# Autodesk Inventor assembly: ARM_012_ArmMount
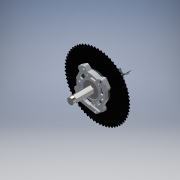
[picture p0: Inventor's stored thumbnail of the model, 180x180]
Saved by Autodesk Inventor 2018.3 (Build 223284000, 284)
## iProperties
Created: 2020-01-31
Part Number: ARM_012_ArmMount
Document SubType Name: Assembly
Designer: 21vogecale
Author: 21vogecale
## Documents named in this file (7)
- C:\Users\21vogecale\Documents\GrabCAD\Infinite Recharge 2020\Build season\ARM_012_ArmMount.iam
- C:\Users\21vogecale\Documents\GrabCAD\Deep Space 2019\Build Season\Brainstorming\End effector (hatches)\_64t_Aluminum_Plate_Sprocket_25_Chain_1-1_8_Bearing_Bore_217-2629.ipt
- C:\Users\21vogecale\Documents\GrabCAD\Deep Space 2019\Build Season\Brainstorming\End effector (hatches)\Arm plastic VersaHub.ipt
- C:\Users\21vogecale\Documents\GrabCAD\Deep Space 2019\Build Season\Chassis\217-2731_0_500_flanged_bearing.ipt
- C:\Users\21vogecale\Documents\GrabCAD\Deep Space 2019\Build Season\Master references\VersaBlock_V2_217-6111.ipt
- C:\Users\21vogecale\Documents\GrabCAD\Deep Space 2019\Build Season\Brainstorming\End effector (hatches)\Arm Pivot Hex Shaft.ipt
- C:\Users\21vogecale\Documents\GrabCAD\Infinite Recharge 2020\Brainstorming\Sam's Brainstorming Folder\Bearing Mount.ipt
## Components (7 placed, 6 different names)
1. _64t_Aluminum_Plate_Sprocket_25_Chain_1-1_8_Bearing_Bore_217-2629:1 — Insert:2, Mate:7, Mate:11
2. Arm plastic VersaHub:1 — Insert:2, Mate:7, Insert:3, Mate:8
3. 217-2731_0_500_flanged_bearing:2 — Mate:5, Mate:6, Mate:10
4. VersaBlock_V2_217-6111:1 — Mate:5, Mate:6, Insert:3, Mate:8
5. Arm Pivot Hex Shaft:1 — Insert:1, Mate:10
6. 217-2731_0_500_flanged_bearing:3 — Mate:1, Mate:2, Insert:1
7. Bearing Mount:1 — Mate:1, Mate:2, Mate:11
## Relationships (11: Mate 8, Insert 3)
- Mate:1: 217-2731_0_500_flanged_bearing:3 ↔ Bearing Mount:1
- Mate:2: 217-2731_0_500_flanged_bearing:3 ↔ Bearing Mount:1
- Mate:5: 217-2731_0_500_flanged_bearing:2 ↔ VersaBlock_V2_217-6111:1
- Mate:6: 217-2731_0_500_flanged_bearing:2 ↔ VersaBlock_V2_217-6111:1
- Insert:1: Arm Pivot Hex Shaft:1 ↔ 217-2731_0_500_flanged_bearing:3
- Insert:2: _64t_Aluminum_Plate_Sprocket_25_Chain_1-1_8_Bearing_Bore_217-2629:1 ↔ Arm plastic VersaHub:1
- Mate:7: _64t_Aluminum_Plate_Sprocket_25_Chain_1-1_8_Bearing_Bore_217-2629:1 ↔ Arm plastic VersaHub:1
- Insert:3: Arm plastic VersaHub:1 ↔ VersaBlock_V2_217-6111:1
- Mate:8: Arm plastic VersaHub:1 ↔ VersaBlock_V2_217-6111:1
- Mate:10: 217-2731_0_500_flanged_bearing:2 ↔ Arm Pivot Hex Shaft:1
- Mate:11 (4.7625 mm): _64t_Aluminum_Plate_Sprocket_25_Chain_1-1_8_Bearing_Bore_217-2629:1 ↔ Bearing Mount:1
